# Autodesk Inventor assembly: ZWO-EFWMini+SM2-adapters
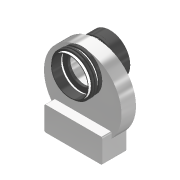
[picture p0: Inventor's stored thumbnail of the model, 180x180]
Saved by Autodesk Inventor 2021 (Build 250183000, 183)
## iProperties
Created: 2022-11-28
Part Number: ZWO-EFWMini+SM2-adapters
Document SubType Name: Assembly
Designer: nvladi
Author: nvladi
## Documents named in this file (5)
- C:\Users\Public\GitHub-public\benchtop-hardware\Benchtop\CAD-model-Inventor2021\library\ZWO-EWF(filter_wheel)\ZWO-EFWMini+SM2-adapters.iam
- C:\Users\Public\GitHub-public\benchtop-hardware\Benchtop\CAD-model-Inventor2021\library\ZWO-EWF(filter_wheel)\ZWO-EFW-Mini.ipt
- C:\Users\Public\GitHub-public\benchtop-hardware\Benchtop\CAD-model-Inventor2021\library\Thorlabs\accessoires\TMA4.ipt
- C:\Users\Public\GitHub-public\benchtop-hardware\Benchtop\CAD-model-Inventor2021\library\Thorlabs\accessoires\SM2T2.ipt
- C:\Users\Public\GitHub-public\benchtop-hardware\Benchtop\CAD-model-Inventor2021\library\Thorlabs\lens_tubes\SM2L05.ipt
## Components (5 placed, 4 different names)
1. ZWO-EFW-Mini:1 — Insert:1, Mate:1
2. TMA4:1 — Insert:1, Mate:2
3. TMA4:2 — Mate:1, Mate:3
4. SM2T2:1 — Mate:2
5. SM2L05:1 — Mate:3
## Relationships (4: Mate 3, Insert 1)
- Insert:1 (-2 mm): ZWO-EFW-Mini:1 ↔ TMA4:1
- Mate:1: ZWO-EFW-Mini:1 ↔ TMA4:2
- Mate:2: TMA4:1 ↔ SM2T2:1
- Mate:3: TMA4:2 ↔ SM2L05:1
